# Autodesk Inventor assembly: Scale Base
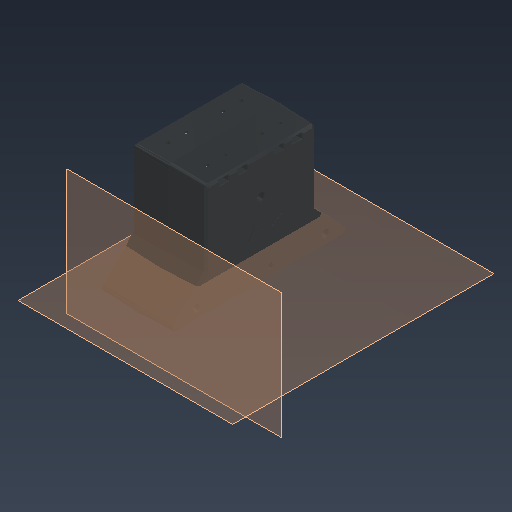
[picture p0: Inventor's stored thumbnail of the model, 512x512]
Saved by Autodesk Inventor 2021 (Build 250183000, 183)
## iProperties
Created: 2021-05-23
Part Number: Scale Base
Document SubType Name: Assembly
Designer: max
Author: max
Revision Number: ANY
## Documents named in this file (8)
- C:\Users\max\Desktop\Vex\TiP FieldCAD\Scales\Scale Base.iam
- C:\Users\max\Desktop\Vex\TiP FieldCAD\Scales\Scale Base.ipt
- C:\Users\max\Desktop\Vex\TiP FieldCAD\Scales\Scale Base Tile Mount.ipt
- C:\Users\max\Desktop\Vex\Library 1.2\Structure\Standoff\Standoff 3.ipt
- C:\Users\max\Desktop\Vex\Library 1.2\Structure\Standoff.ipt
- C:\Users\max\Desktop\Vex\Library 1.2\Structure\Hardware\Screw Steel - Star\Screw 8-32 Steel .500.ipt
- C:\Users\max\Desktop\Vex\Library 1.2\Structure\Hardware\Screw Steel - Star.ipt
- C:\Users\max\Desktop\Vex\Library 1.2\Structure\Hardware\Nut Nylock.ipt
## Components (20 placed, 5 different names)
1. Scale Base:1 — Insert:1, Insert:2, Insert:3, Mate:1, Mate:2, Mate:3, Mate:4, Insert:4, Insert:5, Insert:6, Insert:7, Mate:9, Angle:1, Mate:10, Mate:13, Flush:5
2. Scale Base:2 — Mate:9, Angle:1, Mate:10
3. Standoff 3:1 — Insert:1, Angle:2
4. Standoff 3:2 — Insert:3
5. Standoff 3:3 — Insert:2
6. Screw 8-32 Steel .500:1 — Mate:3, Flush:1, Flush:2
7. Screw 8-32 Steel .500:2 — Mate:2, Flush:2, Mate:4
8. Screw 8-32 Steel .500:3 — Mate:1, Flush:1
9. Nut Nylock:1 — Insert:4
10. Nut Nylock:2 — Insert:5
11. Nut Nylock:3 — Insert:6
12. Nut Nylock:4 — Insert:7
13. Screw 8-32 Steel .500:4
14. Screw 8-32 Steel .500:5
15. Screw 8-32 Steel .500:6
16. Nut Nylock:5
17. Nut Nylock:6
18. Nut Nylock:7
19. Nut Nylock:8
20. Scale Base Tile Mount:1 — Mate:13, Angle:2, Flush:5
## Relationships (29: Insert 11, Mate 11, Flush 5, Angle 2)
- Insert:1: Scale Base:1 ↔ Standoff 3:1
- Insert:2: Scale Base:1 ↔ Standoff 3:3
- Insert:3: Scale Base:1 ↔ Standoff 3:2
- Mate:1: Scale Base:1 ↔ Screw 8-32 Steel .500:3
- Mate:2: Scale Base:1 ↔ Screw 8-32 Steel .500:2
- Mate:3: Scale Base:1 ↔ Screw 8-32 Steel .500:1
- Flush:1: Screw 8-32 Steel .500:1 ↔ Screw 8-32 Steel .500:3
- Flush:2: Screw 8-32 Steel .500:1 ↔ Screw 8-32 Steel .500:2
- Mate:4: Scale Base:1 ↔ Screw 8-32 Steel .500:2
- Insert:4: Scale Base:1 ↔ Nut Nylock:1
- Insert:5: Scale Base:1 ↔ Nut Nylock:2
- Insert:6: Scale Base:1 ↔ Nut Nylock:3
- Insert:7: Scale Base:1 ↔ Nut Nylock:4
- [Mate]: Scale Base:2 ↔ Screw 8-32 Steel .500:6
- [Mate]: Scale Base:2 ↔ Screw 8-32 Steel .500:5
- [Mate]: Scale Base:2 ↔ Screw 8-32 Steel .500:4
- [Flush]: Screw 8-32 Steel .500:4 ↔ Screw 8-32 Steel .500:6
- [Flush]: Screw 8-32 Steel .500:4 ↔ Screw 8-32 Steel .500:5
- [Mate]: Scale Base:2 ↔ Screw 8-32 Steel .500:5
- [Insert]: Scale Base:2 ↔ Nut Nylock:5
- [Insert]: Scale Base:2 ↔ Nut Nylock:6
- [Insert]: Scale Base:2 ↔ Nut Nylock:7
- [Insert]: Scale Base:2 ↔ Nut Nylock:8
- Mate:9: Scale Base:1 ↔ Scale Base:2
- Angle:1 (180 deg): Scale Base:1 ↔ Scale Base:2
- Mate:10: Scale Base:1 ↔ Scale Base:2
- Mate:13: Scale Base:1 ↔ Scale Base Tile Mount:1
- Angle:2 (180 deg): Standoff 3:1 ↔ Scale Base Tile Mount:1
- Flush:5 (-50 mm): Scale Base:1 ↔ Scale Base Tile Mount:1
## Named parameters: d13_d12 = 0 mm, d14_d9 = 0 mm, d15_d10 = 0 mm, d16_d11 = 0 mm, d17_d3 = 0 mm, d18_d4 = 0 mm, d19_d5 = 0 mm, d20_d6 = 0 mm, d21_d7 = 0 mm, d22_d8 = 0 mm
